# Autodesk Inventor assembly: node
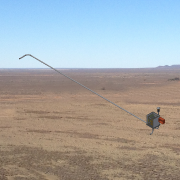
[picture p0: Inventor's stored thumbnail of the model, 180x180]
Saved by Autodesk Inventor 2014 SP1 (Build 180222100, 222)
## iProperties
Created: 2014-03-11
Part Number: node
Document SubType Name: Assembly
Designer: Dave
Author: Dave
## Documents named in this file (14)
- C:\Users\Dave\Desktop\hera-cad\Node\node.iam
- C:\Users\Dave\Desktop\hera-cad\Node\plinth.ipt
- C:\Users\Dave\Desktop\hera-cad\Node\housing.ipt
- C:\Users\Dave\Desktop\hera-cad\Node\snap.ipt
- C:\Users\Dave\Desktop\hera-cad\Node\Acopian-M13-Case.iam
- C:\Users\Dave\Desktop\hera-cad\Node\undergroundPipe.iam
- C:\Users\Dave\Desktop\hera-cad\Node\dcps_mcpc.ipt
- C:\Users\Dave\Desktop\hera-cad\Node\Ground.ipt
- C:\Users\Dave\Desktop\hera-cad\Node\ductFan.ipt
- C:\Users\Dave\Desktop\hera-cad\Node\filter.ipt
- C:\Users\Dave\Desktop\hera-cad\Node\chimneyCap.ipt
- C:\Users\Dave\Desktop\hera-cad\Node\frameAssembly.iam
- C:\Users\Dave\Desktop\hera-cad\Node\pam.ipt
- C:\Users\Dave\Desktop\hera-cad\Node\housingLibAssembly.iam
## Components (36 placed, 13 different names)
1. plinth:1 — Mate:1, Mate:7, Insert:4, toPlinth
2. housing:1 — Mate:1, Mate:6, Mate:9, Mate:13, Mate:21, Flush:8
3. dcps_mcpc:1 — Mate:6
4. undergroundPipe:1 [sub-assembly] — Insert:1, Insert:4
5. Ground:1 — Mate:7
6. ductFan:1 — Insert:1, Insert:2
7. filter:1 — Insert:2, Insert:3
8. chimneyCap:1 — Insert:3
9. frameAssembly:1 [sub-assembly] — Mate:14, Flush:5, Mate:15, Mate:16, Flush:6, Mate:17, Mate:18, Flush:7, Mate:19, toPlinth
10. housingLibAssembly:1 [sub-assembly] — Mate:9
11. pam:1 — Mate:16, Flush:6, Mate:17
12. pam:2
13. pam:3
14. pam:4
15. pam:5
16. pam:6
17. pam:7
18. pam:8
19. pam:9
20. pam:10 — Mate:14, Flush:5, Mate:15
21. pam:11
22. pam:12
23. pam:13
24. pam:14
25. pam:15
26. pam:16
27. pam:17
28. pam:18
29. snap:1 — Mate:18, Flush:7, Mate:19
30. snap:2
31. snap:3
32. snap:4
33. snap:5
34. snap:6
35. Acopian-M13-Case:1 [sub-assembly] — Mate:13, Mate:21, Flush:8
36. Acopian-M13-Case:2 [sub-assembly]
## Component patterns: pam2 (9 elements), pam1 (9 elements), snap (6 elements), analogPower (2 elements)
## Relationships (21: Mate 13, Insert 4, Flush 4)
- Mate:1: plinth:1 ↔ housing:1
- Mate:6: housing:1 ↔ dcps_mcpc:1
- Mate:7: plinth:1 ↔ Ground:1
- Insert:1: undergroundPipe:1 ↔ ductFan:1
- Insert:2: ductFan:1 ↔ filter:1
- Insert:3: filter:1 ↔ chimneyCap:1
- Mate:9: housing:1 ↔ housingLibAssembly:1
- Mate:13: housing:1 ↔ Acopian-M13-Case:1
- Insert:4 (-101.6 mm): plinth:1 ↔ undergroundPipe:1
- Mate:14: frameAssembly:1 ↔ pam:10
- Flush:5: frameAssembly:1 ↔ pam:10
- Mate:15 (50.8 mm): frameAssembly:1 ↔ pam:10
- Mate:16: frameAssembly:1 ↔ pam:1
- Flush:6: frameAssembly:1 ↔ pam:1
- Mate:17 (50.8 mm): frameAssembly:1 ↔ pam:1
- Mate:18: frameAssembly:1 ↔ snap:1
- Flush:7: frameAssembly:1 ↔ snap:1
- Mate:19 (76.2 mm): frameAssembly:1 ↔ snap:1
- toPlinth [Mate]: plinth:1 ↔ frameAssembly:1
- Mate:21 (203.2 mm): housing:1 ↔ Acopian-M13-Case:1
- Flush:8 (406.4 mm): housing:1 ↔ Acopian-M13-Case:1
